# Autodesk Inventor assembly: 40TShaft
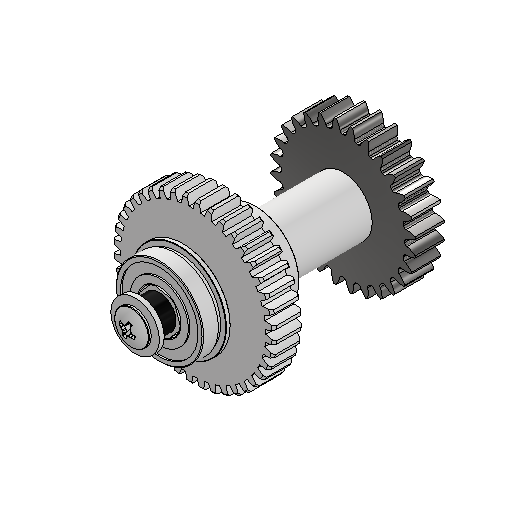
[picture p0: Inventor's stored thumbnail of the model, 512x512]
Saved by Autodesk Inventor 2025 (Build 290162000, 162)
## iProperties
Created: 2024-06-12
Part Number: 40TShaft
Document SubType Name: Assembly
Designer: seene
Author: seene
## Documents named in this file (10)
- C:\Users\seene\Desktop\Stony Brook\SBRT\RCR_Dexter\Drive\v1\40TShaft.iam
- C:\Users\seene\Desktop\Stony Brook\SBRT\RCR_Dexter\Drive\v1\REV-21-1916.ipt
- C:\Users\seene\Desktop\Stony Brook\SBRT\RCR_Dexter\Drive\v1\Gears\am-4710 40T 20DP 500hex 375 FW.ipt
- C:\Users\seene\Desktop\Stony Brook\SBRT\RCR_Dexter\Drive\v1\HexBearingDrivePlateSapcer.ipt
- C:\Users\seene\Desktop\Stony Brook\SBRT\RCR_Dexter\Drive\v1\91770A830_Extra-Wide Truss Head Phillips Screws.ipt
- C:\Users\seene\Desktop\Stony Brook\SBRT\RCR_Dexter\Drive\v1\2879T1_High-Load Oil-Embedded 863 Bronze Thrust Bearing.ipt
- C:\Users\seene\Desktop\Stony Brook\SBRT\RCR_Dexter\Drive\v1\3inRoundHexShaft.ipt
- C:\Users\seene\Desktop\Stony Brook\SBRT\RCR_Dexter\Drive\v1\Spur Gear (28 teeth).ipt
- C:\Users\seene\Desktop\Stony Brook\SBRT\RCR_Dexter\Drive\v1\am-3948-063 500H x 063IN Spacer.ipt
- C:\Users\seene\Desktop\Stony Brook\SBRT\RCR_Dexter\Drive\v1\HexShaftSpacer2.ipt
## Components (13 placed, 9 different names)
1. REV-21-1916:1 — Mate:1, Mate:3, Mate:4
2. REV-21-1916:2 — Mate:2, Mate:3, Mate:17, Flush:1
3. am-4710 40T 20DP 500hex 375 FW:1 — Mate:1, Mate:2, Mate:4, Mate:24, Mate:25, Mate:26
4. HexBearingDrivePlateSapcer:1 — Mate:8, Mate:9, Mate:16, Mate:19
5. 91770A830_Extra-Wide Truss Head Phillips Screws:1 — Mate:10, Mate:11
6. 2879T1_High-Load Oil-Embedded 863 Bronze Thrust Bearing:1 — Mate:8, Mate:9, Mate:10, Mate:11
7. 91770A830_Extra-Wide Truss Head Phillips Screws:2
8. 2879T1_High-Load Oil-Embedded 863 Bronze Thrust Bearing:2 — Mate:18, Mate:22, Mate:27, Mate:29
9. 3inRoundHexShaft:1 — Mate:16, Mate:17, Mate:18, Mate:19, Flush:1, Mate:20, Mate:21, Mate:29
10. Spur Gear (28 teeth):1 — Mate:20, Mate:21, Mate:22, Mate:28
11. am-3948-063 500H x 063IN Spacer:1 — Mate:23, Mate:24, Mate:26
12. am-3948-063 500H x 063IN Spacer:2 — Mate:23, Mate:25
13. HexShaftSpacer2:1 — Mate:27, Mate:28
## Relationships (25: Mate 24, Flush 1)
- Mate:1: REV-21-1916:1 ↔ am-4710 40T 20DP 500hex 375 FW:1
- Mate:2: REV-21-1916:2 ↔ am-4710 40T 20DP 500hex 375 FW:1
- Mate:3 (-19.05 mm): REV-21-1916:1 ↔ REV-21-1916:2
- Mate:4 (1.5875 mm): REV-21-1916:1 ↔ am-4710 40T 20DP 500hex 375 FW:1
- Mate:8: HexBearingDrivePlateSapcer:1 ↔ 2879T1_High-Load Oil-Embedded 863 Bronze Thrust Bearing:1
- Mate:9: HexBearingDrivePlateSapcer:1 ↔ 2879T1_High-Load Oil-Embedded 863 Bronze Thrust Bearing:1
- Mate:10: 91770A830_Extra-Wide Truss Head Phillips Screws:1 ↔ 2879T1_High-Load Oil-Embedded 863 Bronze Thrust Bearing:1
- Mate:11: 91770A830_Extra-Wide Truss Head Phillips Screws:1 ↔ 2879T1_High-Load Oil-Embedded 863 Bronze Thrust Bearing:1
- [Mate]: 91770A830_Extra-Wide Truss Head Phillips Screws:2 ↔ 2879T1_High-Load Oil-Embedded 863 Bronze Thrust Bearing:2
- [Mate]: 91770A830_Extra-Wide Truss Head Phillips Screws:2 ↔ 2879T1_High-Load Oil-Embedded 863 Bronze Thrust Bearing:2
- Mate:16: HexBearingDrivePlateSapcer:1 ↔ 3inRoundHexShaft:1
- Mate:17: REV-21-1916:2 ↔ 3inRoundHexShaft:1
- Mate:18: 2879T1_High-Load Oil-Embedded 863 Bronze Thrust Bearing:2 ↔ 3inRoundHexShaft:1
- Mate:19: HexBearingDrivePlateSapcer:1 ↔ 3inRoundHexShaft:1
- Flush:1: REV-21-1916:2 ↔ 3inRoundHexShaft:1
- Mate:20: 3inRoundHexShaft:1 ↔ Spur Gear (28 teeth):1
- Mate:21: 3inRoundHexShaft:1 ↔ Spur Gear (28 teeth):1
- Mate:22: 2879T1_High-Load Oil-Embedded 863 Bronze Thrust Bearing:2 ↔ Spur Gear (28 teeth):1
- Mate:23: am-3948-063 500H x 063IN Spacer:1 ↔ am-3948-063 500H x 063IN Spacer:2
- Mate:24: am-4710 40T 20DP 500hex 375 FW:1 ↔ am-3948-063 500H x 063IN Spacer:1
- Mate:25: am-4710 40T 20DP 500hex 375 FW:1 ↔ am-3948-063 500H x 063IN Spacer:2
- Mate:26: am-4710 40T 20DP 500hex 375 FW:1 ↔ am-3948-063 500H x 063IN Spacer:1
- Mate:27: 2879T1_High-Load Oil-Embedded 863 Bronze Thrust Bearing:2 ↔ HexShaftSpacer2:1
- Mate:28: Spur Gear (28 teeth):1 ↔ HexShaftSpacer2:1
- Mate:29: 2879T1_High-Load Oil-Embedded 863 Bronze Thrust Bearing:2 ↔ 3inRoundHexShaft:1
## Named parameters: d12_d10 = 0 mm, d13_d11 = 0 mm, Finish1_Area = 16.6644
note: some values were not read from the file. Shown as the stored number, unit unknown: "Finish1_Area".
